# Autodesk Inventor assembly: cover_final_assembly
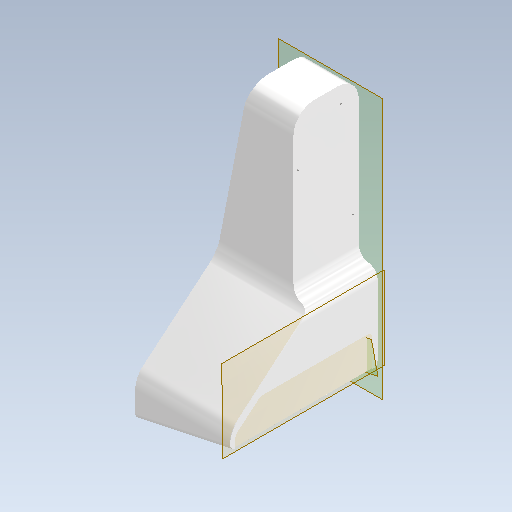
[picture p0: Inventor's stored thumbnail of the model, 512x512]
Saved by Autodesk Inventor 2021 (Build 250183000, 183)
## iProperties
Created: 2021-06-25
Part Number: cover_final_assembly
Document SubType Name: Assembly
Mass: 30077.6 g
Surface Area: 182341 cm^2
Volume: 28275.8 cm^3
Density: 1.06372 g/cm^3
## Documents named in this file (6)
- C:\Users\ocon0143\OneDrive - Flinders\Advn Mech Design Shared\6_Development\2_Design\inventor\cover\cover_final_assembly.iam
- C:\Users\ocon0143\OneDrive - Flinders\Advn Mech Design Shared\6_Development\2_Design\inventor\vehicle_wheelchair\wheelchair\wheelchair_box_extended.ipt
- C:\Users\ocon0143\OneDrive - Flinders\Advn Mech Design Shared\6_Development\2_Design\inventor\cover\cover_open_door.ipt
- C:\Users\ocon0143\OneDrive - Flinders\Advn Mech Design Shared\6_Development\2_Design\inventor\cover\linear_actuator_as.iam
- C:\Users\ocon0143\OneDrive - Flinders\Advn Mech Design Shared\6_Development\2_Design\inventor\cover\cover_inside_support_1.ipt
- \\userOP\O\ocon0143\Documents\Inventor\Content Center Files\R2021\en-US\ISO 4014(2)\ISO 4014 - M8 x 40 - ISO.ipt
## Components (7 placed, 5 different names)
1. wheelchair_box_extended:1 — Mate:1, Flush:1, Flush:2, Mate:2, Flush:3, Mate:3, Mate:4, Flush:4, Flush:5, Mate:6, Mate:7, Mate:8, Mate:9, Mate:10, Mate:11
2. cover_open_door:1 — Mate:2, Flush:3, Mate:5
3. linear_actuator_as:1 [sub-assembly] — Mate:3, Mate:4, Mate:5
4. cover_inside_support_1:1 — Flush:4, Flush:5
5. ISO 4014 M8 x 40:1 — Mate:6, Mate:7
6. ISO 4014 M8 x 40:2 — Mate:8, Mate:9
7. ISO 4014 M8 x 40:3 — Mate:10, Mate:11
## Relationships (16: Mate 11, Flush 5)
- Mate:1: wheelchair_box_extended:1
- Flush:1: wheelchair_box_extended:1
- Flush:2: wheelchair_box_extended:1
- Mate:2: wheelchair_box_extended:1 ↔ cover_open_door:1
- Flush:3 (50 mm): wheelchair_box_extended:1 ↔ cover_open_door:1
- Mate:3: wheelchair_box_extended:1 ↔ linear_actuator_as:1
- Mate:4 (60 mm): wheelchair_box_extended:1 ↔ linear_actuator_as:1
- Mate:5: cover_open_door:1 ↔ linear_actuator_as:1
- Flush:4: wheelchair_box_extended:1 ↔ cover_inside_support_1:1
- Flush:5: wheelchair_box_extended:1 ↔ cover_inside_support_1:1
- Mate:6: wheelchair_box_extended:1 ↔ ISO 4014 M8 x 40:1
- Mate:7: wheelchair_box_extended:1 ↔ ISO 4014 M8 x 40:1
- Mate:8: wheelchair_box_extended:1 ↔ ISO 4014 M8 x 40:2
- Mate:9: wheelchair_box_extended:1 ↔ ISO 4014 M8 x 40:2
- Mate:10: wheelchair_box_extended:1 ↔ ISO 4014 M8 x 40:3
- Mate:11: wheelchair_box_extended:1 ↔ ISO 4014 M8 x 40:3
